# Autodesk Inventor assembly: EFOI-10
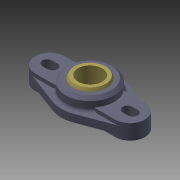
[picture p0: Inventor's stored thumbnail of the model, 180x180]
Saved by Autodesk Inventor 2018 (Build 220112000, 112)
## iProperties
Category: igus Bag
Company: Autodesk, Inc.
Created: 2017-12-12
Part Number: EFOI-10
Document SubType Name: Assembly
Project: FIRST
Catalog Web Link: http://www.igus.com/wpck/5378/igubal_Flanschlager_EFOI?CL=US-en
Description: Flanged spherical bearing
Vendor: igus
Title: Flanged Spherical Bearing
Author: Autodesk, Inc.
Keywords: Black Tote
## Documents named in this file (3)
- D:\FIRST 2018\FIRST 2018 Inventor\FIRST 2018 Black Tote\IGUS Bag\EFOI-10R.iam
- D:\FIRST 2018\FIRST 2018 Inventor\FIRST 2018 Black Tote\IGUS Bag\Parts\EFOI-10_Housing.ipt
- D:\FIRST 2018\FIRST 2018 Inventor\FIRST 2018 Black Tote\IGUS Bag\Parts\EFOI-10_Spherical Bearing.ipt
## Components (2 placed, 2 different names)
1. EFOI-10_Housing:1 — Mate:1
2. EFOI-10_Spherical Bearing:1 — Mate:1
## Relationships (1: Mate 1)
- Mate:1: EFOI-10_Housing:1 ↔ EFOI-10_Spherical Bearing:1
